# Autodesk Inventor assembly: BaseTriangle
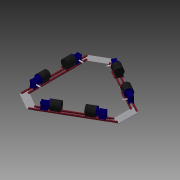
[picture p0: Inventor's stored thumbnail of the model, 180x180]
Saved by Autodesk Inventor 2015 SP1 (Build 190203100, 203)
## iProperties
Created: 2016-04-11
Part Number: BaseTriangle
Document SubType Name: Assembly
Designer: jonesdm
Author: jonesdm
## Documents named in this file (3)
- C:\Users\jonesdm\Desktop\MotionBase\CAD\MotionBaseCAD\Real Platform\BaseTriangle.iam
- C:\Users\jonesdm\Desktop\MotionBase\CAD\MotionBaseCAD\Real Platform\MotorRailSpaced.iam
- C:\Users\jonesdm\Desktop\MotionBase\CAD\MotionBaseCAD\Real Platform\Triangle End2.ipt
## Components (6 placed, 2 different names)
1. MotorRailSpaced:1 [sub-assembly] — Flush:3, Flush:4, Flush:5, Flush:6, Mate:1, Mate:4
2. MotorRailSpaced:2 [sub-assembly] — Flush:1, Flush:2, Flush:7, Flush:8, Mate:2
3. MotorRailSpaced:3 [sub-assembly] — Flush:9, Flush:10, Flush:11, Mate:3
4. Triangle End2:1 — Flush:1, Flush:2, Flush:3, Flush:4, Mate:1, Mate:2
5. Triangle End2:2 — Flush:5, Flush:6, Flush:10, Mate:3, Mate:4
6. Triangle End2:3 — Flush:7, Flush:8, Flush:9, Flush:11
## Relationships (15: Flush 11, Mate 4)
- Flush:1: MotorRailSpaced:2 ↔ Triangle End2:1
- Flush:2: MotorRailSpaced:2 ↔ Triangle End2:1
- Flush:3: MotorRailSpaced:1 ↔ Triangle End2:1
- Flush:4: MotorRailSpaced:1 ↔ Triangle End2:1
- Flush:5: MotorRailSpaced:1 ↔ Triangle End2:2
- Flush:6: MotorRailSpaced:1 ↔ Triangle End2:2
- Flush:7: MotorRailSpaced:2 ↔ Triangle End2:3
- Flush:8: MotorRailSpaced:2 ↔ Triangle End2:3
- Flush:9: MotorRailSpaced:3 ↔ Triangle End2:3
- Flush:10: MotorRailSpaced:3 ↔ Triangle End2:2
- Flush:11: MotorRailSpaced:3 ↔ Triangle End2:3
- Mate:1 (-26.0096 mm): MotorRailSpaced:1 ↔ Triangle End2:1
- Mate:2 (-26.0096 mm): MotorRailSpaced:2 ↔ Triangle End2:1
- Mate:3 (26.0096 mm): MotorRailSpaced:3 ↔ Triangle End2:2
- Mate:4 (-26.0096 mm): MotorRailSpaced:1 ↔ Triangle End2:2
